# Autodesk Inventor assembly: Jetson nano_fixed
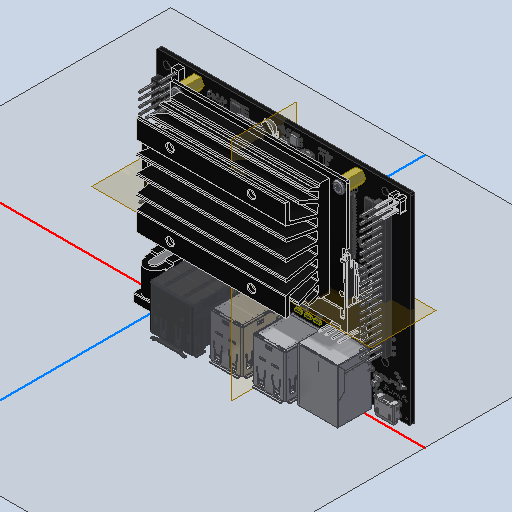
[picture p0: Inventor's stored thumbnail of the model, 512x512]
Saved by Autodesk Inventor 2022 (Build 260153000, 153)
## iProperties
Created: 2019-07-12
Part Number: Jetson nano_fixed
Material: Типовые
Document SubType Name: Assembly
Designer: Петров Иван
Mass: 264.912 g
Surface Area: 866.729 cm^2
Volume: 50.2984 cm^3
Density: 5.26681 g/cm^3
Sending System: Autodesk Translation Framework v8.2.0.1029
Preprocessor: ST-DEVELOPER v18
Title: C:/Users/Toby/Desktop/Jetson nano_fixed.step
## Documents named in this file (6)
- D:\IVAN\Ivan_desktop\Kvantorium\Projects\YouBotRobot\design\standart_components\JetsonNano\Jetson nano_fixed.iam
- D:\IVAN\Ivan_desktop\Kvantorium\Projects\YouBotRobot\design\standart_components\JetsonNano\142-13449-1000-A02_ASM.iam
- D:\IVAN\Ivan_desktop\Kvantorium\Projects\YouBotRobot\design\standart_components\JetsonNano\PORG_HEX_STANDOFF.ipt
- D:\IVAN\Ivan_desktop\Kvantorium\Projects\YouBotRobot\design\standart_components\JetsonNano\PORG_SYSTEM_SCREW.ipt
- D:\IVAN\Ivan_desktop\Kvantorium\Projects\YouBotRobot\design\standart_components\JetsonNano\244-63448-0000-000_ASM.iam
- D:\IVAN\Ivan_desktop\Kvantorium\Projects\YouBotRobot\design\standart_components\JetsonNano\155-0576-000.ipt
## Components (9 placed, 5 different names)
1. 142-13449-1000-A02_ASM:1 [sub-assembly] — Mate:1, Angle:1, Mate:2, Angle:2
2. PORG_HEX_STANDOFF:1
3. PORG_HEX_STANDOFF:2
4. PORG_SYSTEM_SCREW:1
5. PORG_SYSTEM_SCREW:2
6. 244-63448-0000-000_ASM:1 [sub-assembly]
7. PORG_SYSTEM_SCREW:3
8. PORG_SYSTEM_SCREW:4
9. 155-0576-000:1
## Relationships (4: Mate 2, Angle 2)
- Mate:1: 142-13449-1000-A02_ASM:1
- Angle:1 (0 deg): 142-13449-1000-A02_ASM:1
- Mate:2: 142-13449-1000-A02_ASM:1
- Angle:2 (0 deg): 142-13449-1000-A02_ASM:1
